# Autodesk Inventor assembly: ABD_Version 1.0
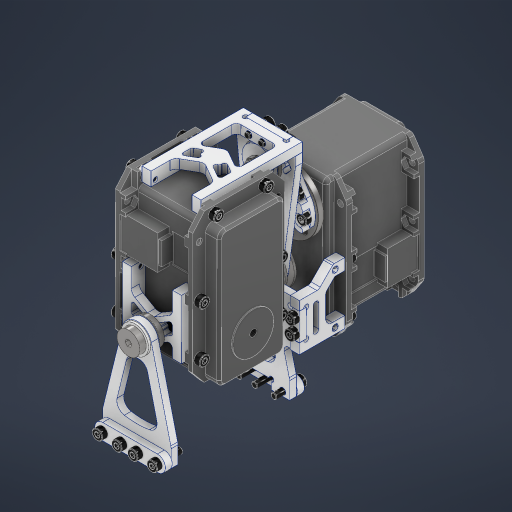
[picture p0: Inventor's stored thumbnail of the model, 512x512]
Saved by Autodesk Inventor 2024.3 (Build 283343000, 343)
## iProperties
Created: 2024-01-25
Part Number: ABD_Version 1.0
Document SubType Name: Assembly
Designer: ASUS
Author: ASUS
## Documents named in this file (6)
- C:\Users\ASUS\Desktop\test\v2_Frame\ABD_V2_Right_OP.iam
- C:\Users\ASUS\Desktop\test\v2_Frame\ABD_MX_64_Roll_Fixation_Set.iam
- C:\Users\ASUS\Desktop\test\v2_Frame\Roll_Fixation_Set.iam
- C:\Users\ASUS\Desktop\test\v2_Frame\ABD_MX_64_Slider_Fixation_Set_Left2Horn.iam
- C:\Users\ASUS\Desktop\test\v2_Frame\ABD_Slider_Set_v2.iam
- C:\Users\ASUS\Desktop\test\v2_Frame\Crank_Slider_Fixer.iam
## Components (5 placed, 5 different names)
1. ABD_MX_64_Roll_Fixation_Set:1 [sub-assembly] — 각도:1
2. Roll_Fixation_Set:1 [sub-assembly] — 메이트:8, 각도:1
3. ABD_MX_64_Slider_Fixation_Set_Left2Horn:1 [sub-assembly] — 메이트:7, 메이트:9
4. ABD_Slider_Set_v2:1 [sub-assembly] — 메이트:8
5. Crank_Slider_Fixer:1 [sub-assembly] — 메이트:7, 메이트:9
## Relationships (9: Mate 6, Insert 2, Angle 1)
- [Insert]: ABD_MX_64_Roll_Fixation_Set:1 ↔ Roll_Fixation_Set:1
- [Mate]: ABD_MX_64_Roll_Fixation_Set:1 ↔ ABD_MX_64_Slider_Fixation_Set_Left2Horn:1
- [Mate]: ABD_MX_64_Roll_Fixation_Set:1 ↔ ABD_MX_64_Slider_Fixation_Set_Left2Horn:1
- [Mate] (0.05 mm): ABD_MX_64_Roll_Fixation_Set:1 ↔ ABD_MX_64_Slider_Fixation_Set_Left2Horn:1
- [Insert]: ABD_Slider_Set_v2:1 ↔ Crank_Slider_Fixer:1
- 메이트:7 [Mate]: ABD_MX_64_Slider_Fixation_Set_Left2Horn:1 ↔ Crank_Slider_Fixer:1
- 메이트:8 [Mate]: Roll_Fixation_Set:1 ↔ ABD_Slider_Set_v2:1
- 각도:1 [Angle] (0 deg): ABD_MX_64_Roll_Fixation_Set:1 ↔ Roll_Fixation_Set:1
- 메이트:9 [Mate]: ABD_MX_64_Slider_Fixation_Set_Left2Horn:1 ↔ Crank_Slider_Fixer:1
## Named parameters: d191_d198 = 0 mm, d192_d199 = 0 mm, d193_d200 = 0.05 mm
